# Autodesk Inventor assembly: puertas
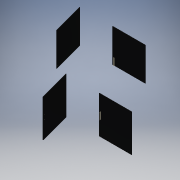
[picture p0: Inventor's stored thumbnail of the model, 180x180]
Saved by Autodesk Inventor 2016 (Build 200138000, 138)
## iProperties
Created: 2015-11-25
Part Number: puertas
Document SubType Name: Assembly
Designer: Daniela
Author: Daniela
## Documents named in this file (4)
- D:\Documents\Carrera\11.Semeste_II_2015\Computacion_grafica\Proyecto\COCINA_FINAL\Cocina\puertas2.iam
- D:\Documents\Carrera\11.Semeste_II_2015\Computacion_grafica\Proyecto\COCINA_FINAL\Cocina\manija.ipt
- D:\Documents\Carrera\11.Semeste_II_2015\Computacion_grafica\Proyecto\COCINA_FINAL\Cocina\puerta_inf2.ipt
- D:\Documents\Carrera\11.Semeste_II_2015\Computacion_grafica\Proyecto\COCINA_FINAL\Cocina\puerta_sup2.ipt
## Components (6 placed, 3 different names)
1. puerta_inf2:1 — Coincidencia:1, Coincidencia:2, Coincidencia:3, Coincidencia:4, Coincidencia:5, Coincidencia:6, Nivelación:1, Coincidencia:7, Nivelación:2
2. manija:1 — Coincidencia:4, Coincidencia:5, Coincidencia:6
3. manija:2 — Coincidencia:1, Coincidencia:2, Coincidencia:3
4. puerta_sup2:1 — Nivelación:1, Coincidencia:7, Nivelación:2, Coincidencia:8, Coincidencia:9, Coincidencia:10, Coincidencia:11, Coincidencia:12, Coincidencia:13
5. manija:3 — Coincidencia:11, Coincidencia:12, Coincidencia:13
6. manija:4 — Coincidencia:8, Coincidencia:9, Coincidencia:10
## Relationships (15: Mate 13, Flush 2)
- Coincidencia:1 [Mate]: puerta_inf2:1 ↔ manija:2
- Coincidencia:2 [Mate]: puerta_inf2:1 ↔ manija:2
- Coincidencia:3 [Mate]: puerta_inf2:1 ↔ manija:2
- Coincidencia:4 [Mate]: puerta_inf2:1 ↔ manija:1
- Coincidencia:5 [Mate]: puerta_inf2:1 ↔ manija:1
- Coincidencia:6 [Mate]: puerta_inf2:1 ↔ manija:1
- Nivelación:1 [Flush] (300 mm): puerta_inf2:1 ↔ puerta_sup2:1
- Coincidencia:7 [Mate] (390 mm): puerta_inf2:1 ↔ puerta_sup2:1
- Nivelación:2 [Flush]: puerta_inf2:1 ↔ puerta_sup2:1
- Coincidencia:8 [Mate]: puerta_sup2:1 ↔ manija:4
- Coincidencia:9 [Mate]: puerta_sup2:1 ↔ manija:4
- Coincidencia:10 [Mate]: puerta_sup2:1 ↔ manija:4
- Coincidencia:11 [Mate]: puerta_sup2:1 ↔ manija:3
- Coincidencia:12 [Mate]: puerta_sup2:1 ↔ manija:3
- Coincidencia:13 [Mate]: puerta_sup2:1 ↔ manija:3
